# Autodesk Inventor assembly: Assembly_Cube_Z-Stage_NEMA8_captive_v0
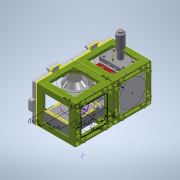
[picture p0: Inventor's stored thumbnail of the model, 180x180]
Saved by Autodesk Inventor 2022 (Build 260153000, 153)
## iProperties
Created: 2020-11-11
Part Number: Assembly_Cube_Z-Stage_NEMA8_captive_v0
Document SubType Name: Assembly
Designer: marsikovabarbora
Author: marsikovabarbora
## Documents named in this file (10)
- G:\My Drive\ASP - M.Sc. Photonics\Practical Modules\MODULE 4 - Master Thesis\2.Experiments\Modules\9.Adjustable_Z_Stage_Module\Manually_driven_MGN12H_Z_Stage\Assembly_Cube_Z-Stage_NEMA8_captive_v0.iam
- G:\My Drive\ASP - M.Sc. Photonics\Practical Modules\MODULE 4 - Master Thesis\2.Experiments\Modules\2.Base_Cube\Base_Cube_IM\Assembly_Cube_empty_IM_v3.iam
- G:\My Drive\ASP - M.Sc. Photonics\Practical Modules\MODULE 4 - Master Thesis\2.Experiments\Modules\9.Adjustable_Z_Stage_Module\Manually_driven_MGN12H_Z_Stage\30_Cube_Z_Focus_MGN_NEMA_rail.ipt
- G:\My Drive\ASP - M.Sc. Photonics\Practical Modules\MODULE 4 - Master Thesis\2.Experiments\Modules\9.Adjustable_Z_Stage_Module\Manually_driven_MGN12H_Z_Stage\00_MGN12H, LINEAR GUIDE BLOCK.ipt
- G:\My Drive\ASP - M.Sc. Photonics\Practical Modules\MODULE 4 - Master Thesis\2.Experiments\Modules\9.Adjustable_Z_Stage_Module\Manually_driven_MGN12H_Z_Stage\30_Cube_Z_Focus_NEMA8_captive_base_v0.ipt
- G:\My Drive\ASP - M.Sc. Photonics\Practical Modules\MODULE 4 - Master Thesis\2.Experiments\Modules\9.Adjustable_Z_Stage_Module\Manually_driven_MGN12H_Z_Stage\00_RS_Pro_Micrometer_small.ipt
- G:\My Drive\ASP - M.Sc. Photonics\Practical Modules\MODULE 4 - Master Thesis\2.Experiments\Modules\9.Adjustable_Z_Stage_Module\Manually_driven_MGN12H_Z_Stage\30_Cube_Z_Focus_NEMA8_captive_micrometerscrewbase_v0.ipt
- G:\My Drive\ASP - M.Sc. Photonics\Practical Modules\MODULE 4 - Master Thesis\2.Experiments\Modules\1.Baseplate\Baseplate_3DP\10_Base_puzzle_v3.ipt
- G:\My Drive\ASP - M.Sc. Photonics\Practical Modules\MODULE 4 - Master Thesis\2.Experiments\Modules\9.Adjustable_Z_Stage_Module\Manually_driven_MGN12H_Z_Stage\00_Microscope_Objective_Lens10x.ipt
- G:\My Drive\ASP - M.Sc. Photonics\Practical Modules\MODULE 4 - Master Thesis\2.Experiments\Modules\9.Adjustable_Z_Stage_Module\Manually_driven_MGN12H_Z_Stage\30_Cube_Cube_Z_Focus_MGN_NEMA_belt_pushing_slide_LONGER_up.ipt
## Components (11 placed, 9 different names)
1. 30_Cube_Z_Focus_MGN_NEMA_rail:1
2. 00_MGN12H, LINEAR GUIDE BLOCK:1 — Rigid:2
3. 30_Cube_Z_Focus_NEMA8_captive_base_v0:1 — Rotational:1, Rotational:2, Rigid:3, Flush:15, Rigid:4
4. 30_Cube_Cube_Z_Focus_MGN_NEMA_belt_pushing_slide_LONGER_up:1 — Rigid:2
5. Assembly_Cube_empty_IM_v3:3 [sub-assembly] — Rigid:3, Flush:15, Rigid:5
6. 00_RS_Pro_Micrometer_small:1 — Rotational:3
7. 30_Cube_Z_Focus_NEMA8_captive_micrometerscrewbase_v0:1 — Rotational:1, Rotational:2, Rotational:3
8. Assembly_Cube_empty_IM_v3:4 [sub-assembly] — Rigid:5, Rotational:4
9. 10_Base_puzzle_v3:1 — Rigid:4, Rigid:6
10. 10_Base_puzzle_v3:2 — Rigid:6
11. 00_Microscope_Objective_Lens10x:1 — Rotational:4
## Relationships (17: Mate 5, WeldJoint 5, RevoluteJoint 4, Flush 2, Angle 1)
- [Mate]: 30_Cube_Z_Focus_MGN_NEMA_rail:1 ↔ 30_Cube_Z_Focus_NEMA8_captive_base_v0:1
- [Mate]: 30_Cube_Z_Focus_MGN_NEMA_rail:1 ↔ 30_Cube_Z_Focus_NEMA8_captive_base_v0:1
- [Mate]: 30_Cube_Z_Focus_MGN_NEMA_rail:1 ↔ 30_Cube_Z_Focus_NEMA8_captive_base_v0:1
- [Flush]: 30_Cube_Z_Focus_MGN_NEMA_rail:1 ↔ 30_Cube_Z_Focus_NEMA8_captive_base_v0:1
- [Mate]: 30_Cube_Z_Focus_MGN_NEMA_rail:1 ↔ 00_MGN12H, LINEAR GUIDE BLOCK:1
- [Mate]: 30_Cube_Z_Focus_MGN_NEMA_rail:1 ↔ 00_MGN12H, LINEAR GUIDE BLOCK:1
- [Angle] (0 deg): 00_MGN12H, LINEAR GUIDE BLOCK:1 ↔ 30_Cube_Cube_Z_Focus_MGN_NEMA_belt_pushing_slide_LONGER_up:1
- Rigid:2 [WeldJoint]: 00_MGN12H, LINEAR GUIDE BLOCK:1 ↔ 30_Cube_Cube_Z_Focus_MGN_NEMA_belt_pushing_slide_LONGER_up:1
- Rotational:1 [RevoluteJoint]: 30_Cube_Z_Focus_NEMA8_captive_base_v0:1 ↔ 30_Cube_Z_Focus_NEMA8_captive_micrometerscrewbase_v0:1
- Rotational:2 [RevoluteJoint]: 30_Cube_Z_Focus_NEMA8_captive_base_v0:1 ↔ 30_Cube_Z_Focus_NEMA8_captive_micrometerscrewbase_v0:1
- Rotational:3 [RevoluteJoint]: 00_RS_Pro_Micrometer_small:1 ↔ 30_Cube_Z_Focus_NEMA8_captive_micrometerscrewbase_v0:1
- Rigid:3 [WeldJoint]: 30_Cube_Z_Focus_NEMA8_captive_base_v0:1 ↔ Assembly_Cube_empty_IM_v3:3
- Flush:15: 30_Cube_Z_Focus_NEMA8_captive_base_v0:1 ↔ Assembly_Cube_empty_IM_v3:3
- Rigid:4 [WeldJoint]: 30_Cube_Z_Focus_NEMA8_captive_base_v0:1 ↔ 10_Base_puzzle_v3:1
- Rigid:5 [WeldJoint]: Assembly_Cube_empty_IM_v3:3 ↔ Assembly_Cube_empty_IM_v3:4
- Rigid:6 [WeldJoint]: 10_Base_puzzle_v3:1 ↔ 10_Base_puzzle_v3:2
- Rotational:4 [RevoluteJoint] (-22 mm): Assembly_Cube_empty_IM_v3:4 ↔ 00_Microscope_Objective_Lens10x:1
